# Autodesk Inventor assembly: UBG-Spulen
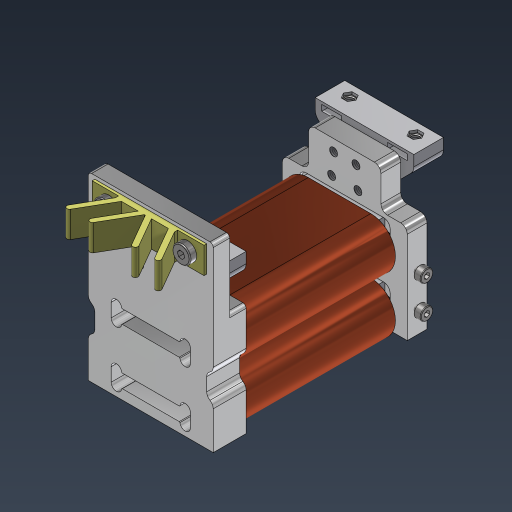
[picture p0: Inventor's stored thumbnail of the model, 512x512]
Saved by Autodesk Inventor 2023.1 (Build 271208000, 208)
## iProperties
Part Number: UBG-Spulen
Material: Generisch
Document SubType Name: Assembly
Designer: rYan
Mass: 307.669 g
Surface Area: 472.647 cm^2
Volume: 59.7033 cm^3
Density: 5.1533 g/cm^3
Author: rYan
## Documents named in this file (8)
- D:\TIGERsGIT\Hardware\mechanik\2024\Inventor\Robot\Kicker\UBG-Spulen.iam
- D:\TIGERsGIT\Hardware\mechanik\2024\Inventor\Robot\Kicker\MG-Spule.iam
- D:\TIGERsGIT\Hardware\mechanik\2024\Inventor\Robot\Kicker\Spulenhalter Hinten.ipt
- D:\TIGERsGIT\Hardware\mechanik\2024\Inventor\Robot\Kicker\Spulenhalter Vorne.ipt
- D:\TIGERsGIT\Hardware\mechanik\2024\Inventor\Robot\Kicker\MG-Kickerboard Winkel.iam
- D:\TIGERsGIT\Hardware\mechanik\2024\Inventor\Inhaltscenter\de-DE\ISO 4762(2)\ISO 4762 - M2 x 6ISO.ipt
- D:\TIGERsGIT\Hardware\mechanik\2024\Inventor\Inhaltscenter\de-DE\DIN 7984\DIN 7984 - M3 x 5.ipt
- D:\TIGERsGIT\Hardware\mechanik\2024\Inventor\Robot\Dribbler\Dribblerdaempfer V2.ipt
## Components (17 placed, 8 different names)
1. MG-Spule:Chip [sub-assembly] — Fluchtend:1, Fluchtend:2, Fluchtend:3, Passend:2, Passend:3, Fluchtend:5, Fluchtend:6
2. MG-Spule:Straight [sub-assembly] — Passend:4, Fluchtend:7, Fluchtend:8
3. Spulenhalter Hinten:1 — Fluchtend:4, Passend:3, Passend:4, Fluchtend:5, Einfügen:12, Passend:7, Einfügen:31, Einfügen:32, Einfügen:33, Einfügen:34
4. Spulenhalter Vorne:1 — Passend:1, Passend:2, Fluchtend:6, Fluchtend:8, Einfügen:11, Passend:6, Einfügen:38, Passend:9
5. MG-Kickerboard Winkel:1 [sub-assembly] — Einfügen:11, Passend:6
6. MG-Kickerboard Winkel:2 [sub-assembly] — Einfügen:12, Passend:7
7. Dribblerdaempfer V2:1 — Einfügen:38, Passend:9, Einfügen:40, Einfügen:41
8. DIN 7984 M3 x 5:3
9. DIN 7984 M3 x 5:4
10. DIN 7984 M3 x 5:5
11. DIN 7984 M3 x 5:6
12. DIN 7984 M3 x 5:1 — Einfügen:41
13. DIN 7984 M3 x 5:2 — Einfügen:40
14. ISO 4762 M2 x 6:1 — Einfügen:32
15. ISO 4762 M2 x 6:2 — Einfügen:31
16. ISO 4762 M2 x 6:3 — Einfügen:33
17. ISO 4762 M2 x 6:4 — Einfügen:34
## Relationships (28: Insert 13, Flush 8, Mate 7)
- Fluchtend:1 [Flush]: MG-Spule:Chip
- Fluchtend:2 [Flush]: MG-Spule:Chip
- Fluchtend:3 [Flush]: MG-Spule:Chip
- Fluchtend:4 [Flush]: Spulenhalter Hinten:1
- Passend:1 [Mate]: Spulenhalter Vorne:1
- Passend:2 [Mate] (0.1 mm): MG-Spule:Chip ↔ Spulenhalter Vorne:1
- Passend:3 [Mate] (0.1 mm): MG-Spule:Chip ↔ Spulenhalter Hinten:1
- Passend:4 [Mate] (0.1 mm): MG-Spule:Straight ↔ Spulenhalter Hinten:1
- Fluchtend:5 [Flush] (-0.25 mm): MG-Spule:Chip ↔ Spulenhalter Hinten:1
- Fluchtend:6 [Flush] (-0.25 mm): MG-Spule:Chip ↔ Spulenhalter Vorne:1
- Fluchtend:7 [Flush]: MG-Spule:Straight
- Fluchtend:8 [Flush] (0.25 mm): MG-Spule:Straight ↔ Spulenhalter Vorne:1
- Einfügen:11 [Insert]: Spulenhalter Vorne:1 ↔ MG-Kickerboard Winkel:1
- Passend:6 [Mate]: Spulenhalter Vorne:1 ↔ MG-Kickerboard Winkel:1
- Einfügen:12 [Insert]: Spulenhalter Hinten:1 ↔ MG-Kickerboard Winkel:2
- Passend:7 [Mate]: Spulenhalter Hinten:1 ↔ MG-Kickerboard Winkel:2
- [Insert]: MG-Kickerboard Winkel:2 ↔ DIN 7984 M3 x 5:6
- [Insert]: MG-Kickerboard Winkel:2 ↔ DIN 7984 M3 x 5:5
- [Insert]: MG-Kickerboard Winkel:1 ↔ DIN 7984 M3 x 5:3
- [Insert]: MG-Kickerboard Winkel:1 ↔ DIN 7984 M3 x 5:4
- Einfügen:31 [Insert] (1 mm): Spulenhalter Hinten:1 ↔ ISO 4762 M2 x 6:2
- Einfügen:32 [Insert] (1 mm): Spulenhalter Hinten:1 ↔ ISO 4762 M2 x 6:1
- Einfügen:33 [Insert] (1 mm): Spulenhalter Hinten:1 ↔ ISO 4762 M2 x 6:3
- Einfügen:34 [Insert] (1 mm): Spulenhalter Hinten:1 ↔ ISO 4762 M2 x 6:4
- Einfügen:38 [Insert]: Spulenhalter Vorne:1 ↔ Dribblerdaempfer V2:1
- Passend:9 [Mate]: Spulenhalter Vorne:1 ↔ Dribblerdaempfer V2:1
- Einfügen:40 [Insert]: Dribblerdaempfer V2:1 ↔ DIN 7984 M3 x 5:2
- Einfügen:41 [Insert]: Dribblerdaempfer V2:1 ↔ DIN 7984 M3 x 5:1
